# Autodesk Inventor assembly: bevelgear_ass
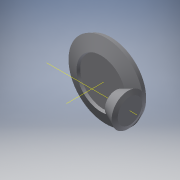
[picture p0: Inventor's stored thumbnail of the model, 180x180]
Saved by Autodesk Inventor 2019 (Build 230136000, 136)
## iProperties
Shininess: 64.0
Angle Display Precision: 2
Document Length Units: 11269
Document Angle Units: 11279
Document Time Units: 11290
Document Mass Units: 11283
Document Length Units Precision: 3
Document Angle Units Precision: 2
Created: 2005-03-17
Part Number: bevelgear_ass
Document SubType Name: Assembly
Designer: Miroslav Petele
Density: 0.0
Volumn: 0.0
Area: 0.0
PropertySet Name: Model Information
Control State: 0
Master: False
Checked Out: False
Author: Miroslav Petele
## Documents named in this file (3)
- C:\Users\Mohamed Teleb\OneDrive - Faculty of Engineering Ain Shams University\Desktop\DOM1STEP\Bevel gearing_PZ1R\Bevel gearing - assembly.iam
- C:\Users\Mohamed Teleb\OneDrive - Faculty of Engineering Ain Shams University\Desktop\DOM1STEP\Bevel gearing_PZ1R\bevelgear_pinion.ipt
- C:\Users\Mohamed Teleb\OneDrive - Faculty of Engineering Ain Shams University\Desktop\DOM1STEP\Bevel gearing_PZ1R\bevelgear_wheel.ipt
## Components (2 placed, 2 different names)
1. bevelgear_pinion:1 — Mate:1, Mate:2
2. bevelgear_wheel:1 — Mate:1, Mate:2
## Relationships (2: Mate 2)
- Mate:1: bevelgear_pinion:1 ↔ bevelgear_wheel:1
- Mate:2: bevelgear_pinion:1 ↔ bevelgear_wheel:1
